# Autodesk Inventor assembly: SPE42 Base Paciente
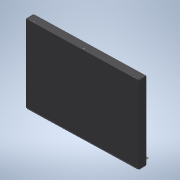
[picture p0: Inventor's stored thumbnail of the model, 180x180]
Saved by Autodesk Inventor 2021.2 (Build 252289000, 289)
## iProperties
Created: 2026-08-25
Part Number: SPE42 Base Paciente
Document SubType Name: Assembly
Designer: nelso
Author: nelso
## Documents named in this file (8)
- C:\Users\nelso\Desktop\Soporte-Paciente-Espinografia\Workspace\SPE42 Base Paciente.iam
- C:\Users\nelso\Desktop\Soporte-Paciente-Espinografia\Workspace\SP26V1 Base Chapa.ipt
- C:\Users\nelso\Desktop\Soporte-Paciente-Espinografia\Workspace\SP32V1 Refuerzo.ipt
- C:\Users\nelso\Desktop\Soporte-Paciente-Espinografia\Workspace\SP40V1 Chapa Base.ipt
- C:\Users\nelso\Desktop\Soporte-Paciente-Espinografia\Workspace\SP41V1 Cubre Base.ipt
- C:\Users\nelso\Desktop\Soporte-Paciente-Espinografia\Workspace\RFPLUS4PO300 Tuerca rem M4 cab red.ipt
- C:\Users\nelso\Desktop\Soporte-Paciente-Espinografia\Workspace\DIN7991M4X0.8L12C.ipt
- C:\Users\nelso\Desktop\Soporte-Paciente-Espinografia\Workspace\SP41V1 Goma Base.ipt
## Components (19 placed, 7 different names)
1. SP26V1 Base Chapa:1
2. SP32V1 Refuerzo:1
3. SP32V1 Refuerzo:2
4. SP32V1 Refuerzo:3
5. SP40V1 Chapa Base:1
6. SP41V1 Cubre Base:1
7. RFPLUS4PO300 Tuerca rem M4 cab red:1
8. RFPLUS4PO300 Tuerca rem M4 cab red:2
9. RFPLUS4PO300 Tuerca rem M4 cab red:3
10. RFPLUS4PO300 Tuerca rem M4 cab red:4
11. RFPLUS4PO300 Tuerca rem M4 cab red:5
12. RFPLUS4PO300 Tuerca rem M4 cab red:6
13. DIN7991M4X0.8L12C:1
14. DIN7991M4X0.8L12C:2
15. DIN7991M4X0.8L12C:3
16. DIN7991M4X0.8L12C:4
17. DIN7991M4X0.8L12C:5
18. DIN7991M4X0.8L12C:6
19. SP41V1 Goma Base:1
## Relationships (42: Mate 30, Flush 12)
- [Mate]: SP26V1 Base Chapa:1 ↔ SP32V1 Refuerzo:2
- [Mate]: SP26V1 Base Chapa:1 ↔ SP32V1 Refuerzo:3
- [Mate]: SP26V1 Base Chapa:1 ↔ SP32V1 Refuerzo:1
- [Mate]: SP26V1 Base Chapa:1 ↔ SP32V1 Refuerzo:3
- [Mate]: SP26V1 Base Chapa:1 ↔ SP32V1 Refuerzo:2
- [Mate]: SP26V1 Base Chapa:1 ↔ SP32V1 Refuerzo:1
- [Flush]: SP26V1 Base Chapa:1 ↔ SP32V1 Refuerzo:2
- [Flush]: SP26V1 Base Chapa:1 ↔ SP32V1 Refuerzo:1
- [Flush]: SP26V1 Base Chapa:1 ↔ SP32V1 Refuerzo:3
- [Mate]: SP26V1 Base Chapa:1 ↔ SP40V1 Chapa Base:1
- [Mate]: SP26V1 Base Chapa:1 ↔ SP40V1 Chapa Base:1
- [Mate]: SP26V1 Base Chapa:1 ↔ SP40V1 Chapa Base:1
- [Flush]: SP26V1 Base Chapa:1 ↔ SP41V1 Cubre Base:1
- [Flush]: SP26V1 Base Chapa:1 ↔ SP41V1 Cubre Base:1
- [Flush] (2 mm): SP26V1 Base Chapa:1 ↔ SP41V1 Cubre Base:1
- [Mate]: SP26V1 Base Chapa:1 ↔ RFPLUS4PO300 Tuerca rem M4 cab red:6
- [Mate]: SP26V1 Base Chapa:1 ↔ RFPLUS4PO300 Tuerca rem M4 cab red:5
- [Mate]: SP26V1 Base Chapa:1 ↔ RFPLUS4PO300 Tuerca rem M4 cab red:4
- [Mate]: SP26V1 Base Chapa:1 ↔ RFPLUS4PO300 Tuerca rem M4 cab red:1
- [Mate]: SP26V1 Base Chapa:1 ↔ RFPLUS4PO300 Tuerca rem M4 cab red:2
- [Mate]: SP26V1 Base Chapa:1 ↔ RFPLUS4PO300 Tuerca rem M4 cab red:3
- [Mate]: SP26V1 Base Chapa:1 ↔ RFPLUS4PO300 Tuerca rem M4 cab red:1
- [Mate]: SP26V1 Base Chapa:1 ↔ RFPLUS4PO300 Tuerca rem M4 cab red:2
- [Mate]: SP26V1 Base Chapa:1 ↔ RFPLUS4PO300 Tuerca rem M4 cab red:3
- [Mate]: SP26V1 Base Chapa:1 ↔ RFPLUS4PO300 Tuerca rem M4 cab red:4
- [Mate]: SP26V1 Base Chapa:1 ↔ RFPLUS4PO300 Tuerca rem M4 cab red:5
- [Mate]: SP26V1 Base Chapa:1 ↔ RFPLUS4PO300 Tuerca rem M4 cab red:6
- [Mate]: SP26V1 Base Chapa:1 ↔ DIN7991M4X0.8L12C:1
- [Mate]: SP26V1 Base Chapa:1 ↔ DIN7991M4X0.8L12C:2
- [Mate]: SP26V1 Base Chapa:1 ↔ DIN7991M4X0.8L12C:3
- [Mate]: SP26V1 Base Chapa:1 ↔ DIN7991M4X0.8L12C:4
- [Mate]: SP26V1 Base Chapa:1 ↔ DIN7991M4X0.8L12C:5
- [Mate]: SP26V1 Base Chapa:1 ↔ DIN7991M4X0.8L12C:6
- [Flush]: SP26V1 Base Chapa:1 ↔ DIN7991M4X0.8L12C:3
- [Flush]: SP26V1 Base Chapa:1 ↔ DIN7991M4X0.8L12C:2
- [Flush]: SP26V1 Base Chapa:1 ↔ DIN7991M4X0.8L12C:1
- [Flush]: SP26V1 Base Chapa:1 ↔ DIN7991M4X0.8L12C:6
- [Flush]: SP26V1 Base Chapa:1 ↔ DIN7991M4X0.8L12C:5
- [Flush]: SP26V1 Base Chapa:1 ↔ DIN7991M4X0.8L12C:4
- [Mate]: SP26V1 Base Chapa:1 ↔ SP41V1 Goma Base:1
- [Mate]: SP26V1 Base Chapa:1 ↔ SP41V1 Goma Base:1
- [Mate]: SP26V1 Base Chapa:1 ↔ SP41V1 Goma Base:1
